# Autodesk Inventor assembly: My Chassy
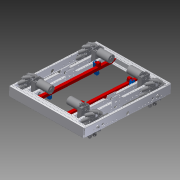
[picture p0: Inventor's stored thumbnail of the model, 180x180]
Saved by Autodesk Inventor 2014 (Build 180170000, 170)
## iProperties
Created: 2016-01-10
Part Number: My Chassy
Document SubType Name: Assembly
Designer: Applefamily
Author: Applefamily
## Documents named in this file (5)
- C:\Users\Applefamily\Documents\Inventor\Strong\Imported Components\My Chassy.iam
- C:\Users\Applefamily\Documents\Inventor\Strong\Imported Components\DriveSide.iam
- C:\Users\Applefamily\Documents\Inventor\Strong\Imported Components\Ground.ipt
- C:\Users\Applefamily\Documents\Inventor\Strong\Imported Components\My2 am-2953 AM14U2 End Sheet Square.ipt.ipt
- My2 am-2953 AM14U2 End Sheet Square.ipt
## Components (5 placed, 3 different names)
1. DriveSide:1 [sub-assembly] — Cylindrical:1, Cylindrical:2, Mate:1, Mate:2, Mate:3, Rotational:1, Rotational:3
2. DriveSide:2 [sub-assembly] — Cylindrical:1, Cylindrical:2, Rotational:2, Rotational:4
3. Ground:1 — Mate:1, Mate:2, Mate:3
4. My2 am-2953 AM14U2 End Sheet Square.ipt:1 — Rotational:1, Rotational:2
5. My2 am-2953 AM14U2 End Sheet Square.ipt:2 — Rotational:3, Rotational:4
## Relationships (9: RevoluteJoint 4, Mate 3, CylindricalJoint 2)
- Cylindrical:1: DriveSide:1 ↔ DriveSide:2
- Cylindrical:2: DriveSide:1 ↔ DriveSide:2
- Mate:1 (101.6 mm): DriveSide:1 ↔ Ground:1
- Mate:2: DriveSide:1 ↔ Ground:1
- Mate:3 (155.1432 mm): DriveSide:1 ↔ Ground:1
- Rotational:1 [RevoluteJoint]: DriveSide:1 ↔ My2 am-2953 AM14U2 End Sheet Square.ipt:1
- Rotational:2 [RevoluteJoint]: DriveSide:2 ↔ My2 am-2953 AM14U2 End Sheet Square.ipt:1
- Rotational:3 [RevoluteJoint]: DriveSide:1 ↔ My2 am-2953 AM14U2 End Sheet Square.ipt:2
- Rotational:4 [RevoluteJoint]: DriveSide:2 ↔ My2 am-2953 AM14U2 End Sheet Square.ipt:2
